# Autodesk Inventor assembly: Wheel_2D
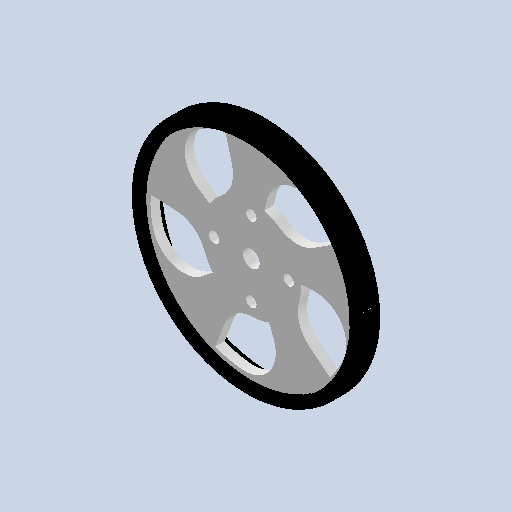
[picture p0: Inventor's stored thumbnail of the model, 512x512]
Saved by Autodesk Inventor 2023 (Build 270158000, 158)
## iProperties
Created: 2024-08-05
Part Number: Wheel_2D
Document SubType Name: Assembly
Designer: LEGION
Author: LEGION
## Documents named in this file (3)
- E:\8 IDEX Pedro P. Diaz\4_Capacitaciones\2_Inventor\Wheel_2D.iam
- E:\8 IDEX Pedro P. Diaz\4_Capacitaciones\2_Inventor\Wheel_2D_Int.ipt
- E:\8 IDEX Pedro P. Diaz\4_Capacitaciones\2_Inventor\Neumatico.ipt
## Components (2 placed, 2 different names)
1. Wheel_2D_Int:1 — Mate:1, Mate:2
2. Neumatico:1 — Mate:1, Mate:2
## Relationships (2: Mate 2)
- Mate:1: Wheel_2D_Int:1 ↔ Neumatico:1
- Mate:2 (0.1 mm): Wheel_2D_Int:1 ↔ Neumatico:1
